# Autodesk Inventor assembly: am-2235a Snow Blower Motor With Hex Shaft
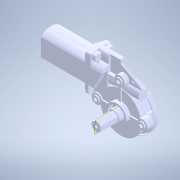
[picture p0: Inventor's stored thumbnail of the model, 180x180]
Saved by Autodesk Inventor 2020.2 (Build 242310000, 310)
## iProperties
Created: 2019-10-31
Part Number: am-2235a Snow Blower Motor With Hex Shaft
Description: STEP AP214
Document SubType Name: Assembly
Designer: robst
Sending System: SolidWorks 2019
Preprocessor: SwSTEP 2.0
Title: am-2235a Snow Blower Motor With Hex Shaft.STEP
Revision Number: ANY
## Documents named in this file (6)
- C:\git\CAD-Development\robSteele\2020BallTriggerMechanism\am-2235a Snow Blower Motor With Hex Shaft.iam
- C:\git\CAD-Development\robSteele\2020BallTriggerMechanism\AM-2235 gearbox housing.ipt
- C:\git\CAD-Development\robSteele\2020BallTriggerMechanism\AM-2235 gear cap.ipt
- C:\git\CAD-Development\robSteele\2020BallTriggerMechanism\AM-2235 motor.ipt
- C:\git\CAD-Development\robSteele\2020BallTriggerMechanism\AM-2235 threaded insert.ipt
- C:\git\CAD-Development\robSteele\2020BallTriggerMechanism\AM-2235a hex output shaft.ipt
## Components (7 placed, 7 different names)
1. AM-2235 gearbox housing_1
2. AM-2235 gear cap_2
3. AM-2235 motor_3
4. AM-2235 threaded insert_4
5. AM-2235 threaded insert_5
6. AM-2235 threaded insert_6
7. AM-2235a hex output shaft_7 — Flush:1, Mate:1
## Relationships (4: Flush 2, Mate 1, Angle 1)
- Flush:1 (-6.35 mm): AM-2235a hex output shaft_7
- Mate:1: AM-2235a hex output shaft_7
- Angle:1 (90 deg)
- Flush:2 (6.35 mm)
